# Autodesk Inventor assembly: F4BSS 20M-YTPSS
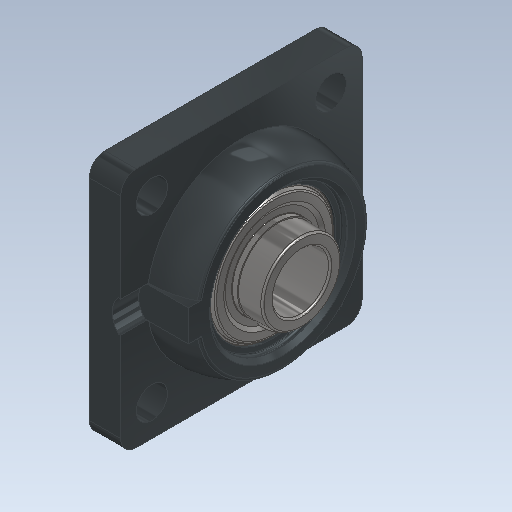
[picture p0: Inventor's stored thumbnail of the model, 512x512]
Saved by Autodesk Inventor 2020 (Build 240168000, 168)
## iProperties
Part Number: F4BSS 20M-YTPSS
Catalog Web Link: www.cadenas.de
Description: AYF_001HC_HH_HY-Y-bearing square flanged units
Vendor: SKF
Document SubType Name: Assembly
Designer: partserver
Manufacturer: SKF
Mass: 680 g
Surface Area: 427.047 cm^2
Volume: 97.3711 cm^3
Density: 6.98359 g/cm^3
Category: PARTsolutions
Company: SKF
PSOL_IDENT_0: {$CADENAS_DATA\23d-libs\skf\bearings_units_and_housings\bearing_units\ball_bearing_units\y-units\ayf
PSOL_IDENT_1: _001hc_hh_hy.prj},201 {VTYP=3D},{STYP=ASSTAB},{NB=F4BSS 20M-YTPSS},{LINA=F4BSS 20M-YTPSS},{NN=AYF_00
PSOL_IDENT_2: 1HC_HH_HY},{DATE=20.08.2020 12:22:38},{GEOMDATE=20.08.2020 12:22:32},{VERSION=},{LINEID=54240},{WBVA
PSOL_IDENT_3: R=COVER},{WBNUMERIC=}  {NB=F4BSS 20M-YTPSS},{LINA=F4BSS 20M-YTPSS},{KT=DUMMY},{DESIGNATION=F4BSS 20M
PSOL_IDENT_4: -YTPSS},{HOUSING=},{BEARING=YAR 204-2LPW/SS},{COVER=},{DD=20},{DDX=},{DDALG=20.000},{DD1=28.200},{DD
PSOL_IDENT_5: 2=MIN},{DD3=},{AALG=25.800},{A=},{AX=},{AXX=25.8},{A1ALG=11.100},{A1=},{A1X=},{A1XX=11.1},{A3ALG=0.0
PSOL_IDENT_6: 00},{A3=},{A3X=},{A5ALG=24.500},{A5=},{A5X=},{A5XX=24.5},{B=31.000},{B1=MIN},{B1X=},{B4ALG=4.500},{B
PSOL_IDENT_7: 4=4.5},{B4X=},{DAAALG=0.000},{DAA=},{DAAX=},{DB=MIN},{DB1=MIN},{DB1X=},{DB2=MIN},{DB2X=},{HA=},{J=MI
PSOL_IDENT_8: N},{JX=},{JXX=63.5},{L=MIN},{LX=},{LXX=85.7},{N=MIN},{NX=},{NXX=11.1},{SS1=18.300},{SS1X=},{T=32.600
PSOL_IDENT_9: },{TX=},{DN=MIN},{SWN=},{GN=},{RG=},{RGX=},{R1=},{R1X=},{J6=},{J7=MIN},{N4=},{D=47.000},{C=14.000},{
PSOL_IDENT_10: R12=0.600},{DW=7.938},{B3=MIN},{PITCH=33.500},{LOAD1=10.800},{LOAD2=6.550},{LOAD3=0.280},{SPEED1=500
PSOL_IDENT_11: 0},{II=1},{Z=8},{MASS=0.680},{MASSX=},{G2=M6x0.75},{HKSGS=3},{RTTGS=4},{ALPHA=},{GALG=10.000},{G=},{
PSOL_IDENT_12: GX=},{GXX=10},{GINALG=0.375},{GIN=},{GINX=},{GINXX=0.375000002475},{EC=},{BS=},{SLEEVE=},{POPULAR=},
PSOL_IDENT_13: {D1=MIN},{K=},{CC1=},{BRGTYP=BBY_006},{COVERALG=  '', 'No end cover' },{SUPPRESSED=unsuppressed},{TC=
PSOL_IDENT_14: F4BSS 20M-YTPSS},{PPATH=y-bearing_square_flanged_units_parts/ayf_001hc_hh_hy_asmtpl.prj}
NB: F4BSS 20M-YTPSS
NN: AYF_001HC_HH_HY
NT: Y-bearing square flanged units
NBSYN: $TC.
LINA: F4BSS 20M-YTPSS
CATALOG: SKF
DESIGNATION: F4BSS 20M-YTPSS
BEARING: YAR 204-2LPW/SS
COVER: No end cover
DDALG: 20
J: 0
L: 0
T: 32.6
LOAD1: 10.8
LOAD2: 6.55
SPEED1: 5000
SUPPLIER: SKF
ARTICLENO: F4BSS 20M-YTPSS
BOMINFO: F4BSS 20M-YTPSS
CREATOR: CADENAS GmbH
Title: F4BSS 20M-YTPSS
Author: Cadenas PARTsolutions
Comments: Y-bearing square flanged units
## Documents named in this file (5)
- C:\Users\Hesekiel\Desktop\Equatorial-Mount-MUM\Mechanika\Mechanizm elewacji Filip\CAD\F4BSS 20M-YTPSS\F4BSS 20M-YTPSS.iam
- C:\Users\Hesekiel\Desktop\Equatorial-Mount-MUM\Mechanika\Mechanizm elewacji Filip\CAD\F4BSS 20M-YTPSS\F4BSS 20M-YTPSS-dummy.ipt
- C:\Users\Hesekiel\Desktop\Equatorial-Mount-MUM\Mechanika\Mechanizm elewacji Filip\CAD\F4BSS 20M-YTPSS\F4BSS 504-Y-housing.ipt
- C:\Users\Hesekiel\Desktop\Equatorial-Mount-MUM\Mechanika\Mechanizm elewacji Filip\CAD\F4BSS 20M-YTPSS\YAR 204-2LPW_SS-28_02014 -bearing.ipt
- C:\Users\Hesekiel\Desktop\Equatorial-Mount-MUM\Mechanika\Mechanizm elewacji Filip\CAD\F4BSS 20M-YTPSS\20-47-31-14-ybrg1-47-7_938-33_5.ipt
## Components (11 placed, 4 different names)
1. F4BSS 20M-YTPSS-dummy:1 — brg_XY@1 <-> housing_XY@2, brg_Z@1 <-> housing_Z@2, brg_YZ@1 <-> housing_YZ@2
2. F4BSS 504-Y-housing:1 — brg_XY@1 <-> housing_XY@2, brg_Z@1 <-> housing_Z@2, brg_YZ@1 <-> housing_YZ@2, housing_XY@2 <-> brg3_XY@3, housing_Z@2 <-> brg3_Z@3, housing_YZ@2 <-> brg3_YZ@3
3. YAR 204-2LPW_SS-28_02014 -bearing:1 — housing_XY@2 <-> brg3_XY@3, housing_Z@2 <-> brg3_Z@3, housing_YZ@2 <-> brg3_YZ@3, ball_1_XY@3 <-> ball_XY@4, ball_1_Z@3 <-> ball_Z@4, ball_1_YZ@3 <-> ball_YZ@4, ball_2_XY@3 <-> ball_XY@5, ball_2_Z@3 <-> ball_Z@5, ball_2_YZ@3 <-> ball_YZ@5, ball_3_XY@3 <-> ball_XY@6, ball_3_Z@3 <-> ball_Z@6, ball_3_YZ@3 <-> ball_YZ@6, ball_4_XY@3 <-> ball_XY@7, ball_4_Z@3 <-> ball_Z@7, ball_4_YZ@3 <-> ball_YZ@7, ball_5_XY@3 <-> ball_XY@8, ball_5_Z@3 <-> ball_Z@8, ball_5_YZ@3 <-> ball_YZ@8, ball_6_XY@3 <-> ball_XY@9, ball_6_Z@3 <-> ball_Z@9, ball_6_YZ@3 <-> ball_YZ@9, ball_7_XY@3 <-> ball_XY@10, ball_7_Z@3 <-> ball_Z@10, ball_7_YZ@3 <-> ball_YZ@10, ball_8_XY@3 <-> ball_XY@11, ball_8_Z@3 <-> ball_Z@11, ball_8_YZ@3 <-> ball_YZ@11
4. 20-47-31-14-ybrg1-47-7_938-33_5:1 — ball_1_XY@3 <-> ball_XY@4, ball_1_Z@3 <-> ball_Z@4, ball_1_YZ@3 <-> ball_YZ@4
5. 20-47-31-14-ybrg1-47-7_938-33_5:2 — ball_2_XY@3 <-> ball_XY@5, ball_2_Z@3 <-> ball_Z@5, ball_2_YZ@3 <-> ball_YZ@5
6. 20-47-31-14-ybrg1-47-7_938-33_5:3 — ball_3_XY@3 <-> ball_XY@6, ball_3_Z@3 <-> ball_Z@6, ball_3_YZ@3 <-> ball_YZ@6
7. 20-47-31-14-ybrg1-47-7_938-33_5:4 — ball_4_XY@3 <-> ball_XY@7, ball_4_Z@3 <-> ball_Z@7, ball_4_YZ@3 <-> ball_YZ@7
8. 20-47-31-14-ybrg1-47-7_938-33_5:5 — ball_5_XY@3 <-> ball_XY@8, ball_5_Z@3 <-> ball_Z@8, ball_5_YZ@3 <-> ball_YZ@8
9. 20-47-31-14-ybrg1-47-7_938-33_5:6 — ball_6_XY@3 <-> ball_XY@9, ball_6_Z@3 <-> ball_Z@9, ball_6_YZ@3 <-> ball_YZ@9
10. 20-47-31-14-ybrg1-47-7_938-33_5:7 — ball_7_XY@3 <-> ball_XY@10, ball_7_Z@3 <-> ball_Z@10, ball_7_YZ@3 <-> ball_YZ@10
11. 20-47-31-14-ybrg1-47-7_938-33_5:8 — ball_8_XY@3 <-> ball_XY@11, ball_8_Z@3 <-> ball_Z@11, ball_8_YZ@3 <-> ball_YZ@11
## Relationships (30: Mate 19, Angle 10, Flush 1)
- brg_XY@1 <-> housing_XY@2 [Mate]: F4BSS 20M-YTPSS-dummy:1 ↔ F4BSS 504-Y-housing:1
- brg_Z@1 <-> housing_Z@2 [Mate]: F4BSS 20M-YTPSS-dummy:1 ↔ F4BSS 504-Y-housing:1
- brg_YZ@1 <-> housing_YZ@2 [Angle] (180 deg): F4BSS 20M-YTPSS-dummy:1 ↔ F4BSS 504-Y-housing:1
- housing_XY@2 <-> brg3_XY@3 [Flush] (32.6 mm): F4BSS 504-Y-housing:1 ↔ YAR 204-2LPW_SS-28_02014 -bearing:1
- housing_Z@2 <-> brg3_Z@3 [Mate]: F4BSS 504-Y-housing:1 ↔ YAR 204-2LPW_SS-28_02014 -bearing:1
- housing_YZ@2 <-> brg3_YZ@3 [Angle] (0 deg): F4BSS 504-Y-housing:1 ↔ YAR 204-2LPW_SS-28_02014 -bearing:1
- ball_1_XY@3 <-> ball_XY@4 [Mate]: YAR 204-2LPW_SS-28_02014 -bearing:1 ↔ 20-47-31-14-ybrg1-47-7_938-33_5:1
- ball_1_Z@3 <-> ball_Z@4 [Mate]: YAR 204-2LPW_SS-28_02014 -bearing:1 ↔ 20-47-31-14-ybrg1-47-7_938-33_5:1
- ball_1_YZ@3 <-> ball_YZ@4 [Angle] (0 deg): YAR 204-2LPW_SS-28_02014 -bearing:1 ↔ 20-47-31-14-ybrg1-47-7_938-33_5:1
- ball_2_XY@3 <-> ball_XY@5 [Mate]: YAR 204-2LPW_SS-28_02014 -bearing:1 ↔ 20-47-31-14-ybrg1-47-7_938-33_5:2
- ball_2_Z@3 <-> ball_Z@5 [Mate]: YAR 204-2LPW_SS-28_02014 -bearing:1 ↔ 20-47-31-14-ybrg1-47-7_938-33_5:2
- ball_2_YZ@3 <-> ball_YZ@5 [Angle] (0 deg): YAR 204-2LPW_SS-28_02014 -bearing:1 ↔ 20-47-31-14-ybrg1-47-7_938-33_5:2
- ball_3_XY@3 <-> ball_XY@6 [Mate]: YAR 204-2LPW_SS-28_02014 -bearing:1 ↔ 20-47-31-14-ybrg1-47-7_938-33_5:3
- ball_3_Z@3 <-> ball_Z@6 [Mate]: YAR 204-2LPW_SS-28_02014 -bearing:1 ↔ 20-47-31-14-ybrg1-47-7_938-33_5:3
- ball_3_YZ@3 <-> ball_YZ@6 [Angle] (0 deg): YAR 204-2LPW_SS-28_02014 -bearing:1 ↔ 20-47-31-14-ybrg1-47-7_938-33_5:3
- ball_4_XY@3 <-> ball_XY@7 [Mate]: YAR 204-2LPW_SS-28_02014 -bearing:1 ↔ 20-47-31-14-ybrg1-47-7_938-33_5:4
- ball_4_Z@3 <-> ball_Z@7 [Mate]: YAR 204-2LPW_SS-28_02014 -bearing:1 ↔ 20-47-31-14-ybrg1-47-7_938-33_5:4
- ball_4_YZ@3 <-> ball_YZ@7 [Angle] (0 deg): YAR 204-2LPW_SS-28_02014 -bearing:1 ↔ 20-47-31-14-ybrg1-47-7_938-33_5:4
- ball_5_XY@3 <-> ball_XY@8 [Mate]: YAR 204-2LPW_SS-28_02014 -bearing:1 ↔ 20-47-31-14-ybrg1-47-7_938-33_5:5
- ball_5_Z@3 <-> ball_Z@8 [Mate]: YAR 204-2LPW_SS-28_02014 -bearing:1 ↔ 20-47-31-14-ybrg1-47-7_938-33_5:5
- ball_5_YZ@3 <-> ball_YZ@8 [Angle] (0 deg): YAR 204-2LPW_SS-28_02014 -bearing:1 ↔ 20-47-31-14-ybrg1-47-7_938-33_5:5
- ball_6_XY@3 <-> ball_XY@9 [Mate]: YAR 204-2LPW_SS-28_02014 -bearing:1 ↔ 20-47-31-14-ybrg1-47-7_938-33_5:6
- ball_6_Z@3 <-> ball_Z@9 [Mate]: YAR 204-2LPW_SS-28_02014 -bearing:1 ↔ 20-47-31-14-ybrg1-47-7_938-33_5:6
- ball_6_YZ@3 <-> ball_YZ@9 [Angle] (0 deg): YAR 204-2LPW_SS-28_02014 -bearing:1 ↔ 20-47-31-14-ybrg1-47-7_938-33_5:6
- ball_7_XY@3 <-> ball_XY@10 [Mate]: YAR 204-2LPW_SS-28_02014 -bearing:1 ↔ 20-47-31-14-ybrg1-47-7_938-33_5:7
- ball_7_Z@3 <-> ball_Z@10 [Mate]: YAR 204-2LPW_SS-28_02014 -bearing:1 ↔ 20-47-31-14-ybrg1-47-7_938-33_5:7
- ball_7_YZ@3 <-> ball_YZ@10 [Angle] (0 deg): YAR 204-2LPW_SS-28_02014 -bearing:1 ↔ 20-47-31-14-ybrg1-47-7_938-33_5:7
- ball_8_XY@3 <-> ball_XY@11 [Mate]: YAR 204-2LPW_SS-28_02014 -bearing:1 ↔ 20-47-31-14-ybrg1-47-7_938-33_5:8
- ball_8_Z@3 <-> ball_Z@11 [Mate]: YAR 204-2LPW_SS-28_02014 -bearing:1 ↔ 20-47-31-14-ybrg1-47-7_938-33_5:8
- ball_8_YZ@3 <-> ball_YZ@11 [Angle] (0 deg): YAR 204-2LPW_SS-28_02014 -bearing:1 ↔ 20-47-31-14-ybrg1-47-7_938-33_5:8
